# Autodesk Inventor assembly: złożenie
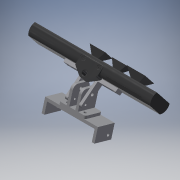
[picture p0: Inventor's stored thumbnail of the model, 180x180]
Saved by Autodesk Inventor 2017 (Build 210142000, 142)
## iProperties
Part Number: złożenie
Material: Ogólny
Document SubType Name: Assembly
Designer: patry
Author: patry
## Documents named in this file (5)
- C:\Users\patry\Desktop\realsens\mocowanie\złożenie.iam
- C:\Users\patry\Desktop\realsens\mocowanie\Część1.ipt
- C:\Users\patry\Desktop\realsens\mocowanie\Część2.ipt
- C:\Users\patry\Desktop\realsens\mocowanie\Część3.ipt
- C:\Users\patry\Desktop\realsens\SR305_peripheral_assembly_external.iam
## Components (4 placed, 4 different names)
1. Część1:1 — Wstaw:3, Wstaw:4, Wstaw:5
2. Część2:1 — Wstaw:1, Wstaw:2
3. Część3:1 — Wstaw:1, Wstaw:2, Wstaw:3
4. SR305_peripheral_assembly_external:1 [sub-assembly] — Wstaw:4, Wstaw:5
## Relationships (5: Insert 5)
- Wstaw:1 [Insert]: Część2:1 ↔ Część3:1
- Wstaw:2 [Insert]: Część2:1 ↔ Część3:1
- Wstaw:3 [Insert]: Część1:1 ↔ Część3:1
- Wstaw:4 [Insert]: Część1:1 ↔ SR305_peripheral_assembly_external:1
- Wstaw:5 [Insert]: Część1:1 ↔ SR305_peripheral_assembly_external:1
